# Autodesk Inventor assembly: Assembly1
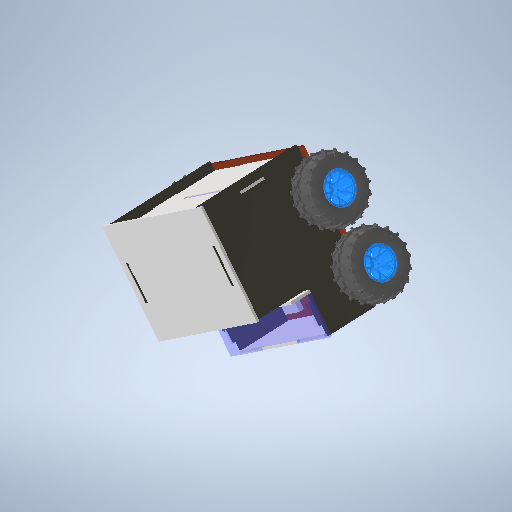
[picture p0: Inventor's stored thumbnail of the model, 512x512]
Saved by Autodesk Inventor 2025.3 (Build 293356030, 356C)
## iProperties
Created: 2026-06-26
Part Number: Assembly1
Document SubType Name: Assembly
Designer: user
Author: user
## Documents named in this file (12)
- C:\Docs\shcool\dojo\Design_2\Assembly1.iam
- C:\Docs\shcool\dojo\Design_2\hood.ipt
- C:\Docs\shcool\dojo\Design_2\side.ipt
- C:\Docs\shcool\dojo\Design_2\top.ipt
- C:\Docs\shcool\dojo\Design_2\back.ipt
- C:\Docs\shcool\dojo\Design_2\base_2.ipt
- C:\Docs\shcool\dojo\Design_1\Hub-12-Eixo6_aluminio.ipt
- C:\Docs\shcool\dojo\Design_1\motor.ipt
- C:\Docs\shcool\dojo\Design_1\Spiked Rubber Wheel 120mm.ipt
- C:\Docs\shcool\dojo\Design_2\cover.ipt
- C:\Docs\shcool\dojo\Design_2\front.ipt
- C:\Docs\shcool\dojo\Design_2\U-bracket.ipt
## Components (24 placed, 11 different names)
1. hood:1 — Mate:42, Mate:43, Mate:47, Mate:49, Mate:71, Mate:72
2. side:1 — Mate:44, Mate:48, Mate:70, Mate:73, Mate:74
3. top:1 — Mate:5, Mate:6
4. side:2 — Mate:5, Mate:6, Mate:7, Mate:8
5. back:1 — Mate:7, Mate:8, Mate:42, Mate:43, Mate:44, Mate:70
6. base_2:1 — Mate:57, Mate:58, Mate:59, Mate:60, Mate:61, Mate:73, Mate:74
7. motor:1 — Insert:3, Mate:63, Mate:68
8. Hub-12-Eixo6_aluminio:2 — Insert:3, Mate:29, Mate:30
9. Spiked Rubber Wheel 120mm:2 — Mate:29, Mate:30
10. front:1 — Mate:71, Mate:72
11. cover:1 — Mate:47, Mate:48, Mate:49
12. motor:2 — Mate:65, Mate:69
13. Hub-12-Eixo6_aluminio:3
14. Spiked Rubber Wheel 120mm:3
15. motor:3 — Mate:62, Mate:67
16. Hub-12-Eixo6_aluminio:4
17. Spiked Rubber Wheel 120mm:4
18. motor:4 — Mate:64, Mate:66
19. Hub-12-Eixo6_aluminio:5
20. Spiked Rubber Wheel 120mm:5
21. U-bracket:1 — Mate:57, Mate:58, Mate:62, Mate:67
22. U-bracket:2 — Mate:60, Mate:65, Mate:69
23. U-bracket:3 — Mate:59, Mate:64, Mate:66
24. U-bracket:4 — Mate:61, Mate:63, Mate:68
## Relationships (40: Mate 36, Insert 4)
- Mate:5: top:1 ↔ side:2
- Mate:6: top:1 ↔ side:2
- Mate:7: side:2 ↔ back:1
- Mate:8: side:2 ↔ back:1
- Insert:3: motor:1 ↔ Hub-12-Eixo6_aluminio:2
- Mate:29: Hub-12-Eixo6_aluminio:2 ↔ Spiked Rubber Wheel 120mm:2
- Mate:30: Hub-12-Eixo6_aluminio:2 ↔ Spiked Rubber Wheel 120mm:2
- Mate:42: hood:1 ↔ back:1
- Mate:43: hood:1 ↔ back:1
- Mate:44: side:1 ↔ back:1
- Mate:47: hood:1 ↔ cover:1
- Mate:48: side:1 ↔ cover:1
- Mate:49: hood:1 ↔ cover:1
- [Insert]: motor:2 ↔ Hub-12-Eixo6_aluminio:3
- [Mate]: Hub-12-Eixo6_aluminio:3 ↔ Spiked Rubber Wheel 120mm:3
- [Mate]: Hub-12-Eixo6_aluminio:3 ↔ Spiked Rubber Wheel 120mm:3
- [Insert]: motor:3 ↔ Hub-12-Eixo6_aluminio:4
- [Mate]: Hub-12-Eixo6_aluminio:4 ↔ Spiked Rubber Wheel 120mm:4
- [Mate]: Hub-12-Eixo6_aluminio:4 ↔ Spiked Rubber Wheel 120mm:4
- [Insert]: motor:4 ↔ Hub-12-Eixo6_aluminio:5
- [Mate]: Hub-12-Eixo6_aluminio:5 ↔ Spiked Rubber Wheel 120mm:5
- [Mate]: Hub-12-Eixo6_aluminio:5 ↔ Spiked Rubber Wheel 120mm:5
- Mate:57: base_2:1 ↔ U-bracket:1
- Mate:58: base_2:1 ↔ U-bracket:1
- Mate:59: base_2:1 ↔ U-bracket:3
- Mate:60: base_2:1 ↔ U-bracket:2
- Mate:61: base_2:1 ↔ U-bracket:4
- Mate:62: motor:3 ↔ U-bracket:1
- Mate:63: motor:1 ↔ U-bracket:4
- Mate:64: motor:4 ↔ U-bracket:3
- Mate:65: motor:2 ↔ U-bracket:2
- Mate:66: motor:4 ↔ U-bracket:3
- Mate:67: motor:3 ↔ U-bracket:1
- Mate:68: motor:1 ↔ U-bracket:4
- Mate:69: motor:2 ↔ U-bracket:2
- Mate:70: side:1 ↔ back:1
- Mate:71: hood:1 ↔ front:1
- Mate:72: hood:1 ↔ front:1
- Mate:73: side:1 ↔ base_2:1
- Mate:74: side:1 ↔ base_2:1
## Named parameters: d85_d39 = 0 mm, d86_d47 = 0 mm, d87_d48 = 0 mm, d88_d39 = 0 mm, d89_d47 = 0 mm, d90_d48 = 0 mm, d91_d39 = 0 mm, d92_d47 = 0 mm, d93_d48 = 0 mm
